# Autodesk Inventor assembly: GGC_V1
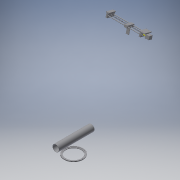
[picture p0: Inventor's stored thumbnail of the model, 180x180]
Saved by Autodesk Inventor 2016 (Build 200138000, 138)
## iProperties
Created: 2016-04-14
Part Number: GGC_V1
Document SubType Name: Assembly
Designer: rmarkowi
Author: rmarkowi
## Documents named in this file (11)
- C:\Users\rmarkowi\Documents\GGC\V1\GGC_V1.iam
- C:\Users\rmarkowi\Documents\GGC\V1\Inner Pole.ipt
- C:\Users\rmarkowi\Documents\GGC\V1\Turntable_2.ipt
- C:\Users\rmarkowi\Documents\GGC\V1\Near Gantry Bracket.ipt
- C:\Users\rmarkowi\Documents\GGC\V1\Threaded Rod.ipt
- C:\Users\rmarkowi\Documents\GGC\V1\Unthreaded Rod.ipt
- C:\Users\rmarkowi\Documents\GGC\V1\Far Gantry Bracket.ipt
- C:\Users\rmarkowi\Documents\GGC\V1\Traveller.ipt
- C:\Users\rmarkowi\Documents\GGC\V1\Threaded Rod Nut.ipt
- C:\Users\rmarkowi\Documents\GGC\V1\Threaded Rod Coupler.ipt
- C:\Users\rmarkowi\Documents\GGC\V1\NEMA23 Motor.ipt
## Components (12 placed, 10 different names)
1. Inner Pole:1
2. Turntable_2:1
3. Threaded Rod:1 — Mate:8, Mate:9, Mate:21
4. Unthreaded Rod:1 — Mate:10, Mate:11, Mate:18
5. Unthreaded Rod:2 — Mate:6, Mate:7, Mate:19, Flush:1, Mate:24
6. Near Gantry Bracket:2 — Flush:1, Flush:2, Mate:24, Mate:25, Mate:26
7. Far Gantry Bracket:1 — Mate:6, Mate:7, Mate:8, Mate:9, Mate:10, Mate:11, Flush:2
8. Traveller:1 — Mate:12, Mate:13, Mate:14, Mate:15, Mate:16, Mate:17, Mate:18, Mate:19
9. Threaded Rod Nut:1 — Mate:12, Mate:13, Mate:14
10. Threaded Rod Nut:2 — Mate:15, Mate:16, Mate:17
11. Threaded Rod Coupler:1 — Mate:21, Mate:22, Mate:23
12. NEMA23 Motor:1 — Mate:22, Mate:23, Mate:25, Mate:26
## Relationships (22: Mate 20, Flush 2)
- Mate:6: Unthreaded Rod:2 ↔ Far Gantry Bracket:1
- Mate:7: Unthreaded Rod:2 ↔ Far Gantry Bracket:1
- Mate:8: Threaded Rod:1 ↔ Far Gantry Bracket:1
- Mate:9: Threaded Rod:1 ↔ Far Gantry Bracket:1
- Mate:10: Unthreaded Rod:1 ↔ Far Gantry Bracket:1
- Mate:11: Unthreaded Rod:1 ↔ Far Gantry Bracket:1
- Mate:12: Traveller:1 ↔ Threaded Rod Nut:1
- Mate:13: Traveller:1 ↔ Threaded Rod Nut:1
- Mate:14: Traveller:1 ↔ Threaded Rod Nut:1
- Mate:15: Traveller:1 ↔ Threaded Rod Nut:2
- Mate:16: Traveller:1 ↔ Threaded Rod Nut:2
- Mate:17: Traveller:1 ↔ Threaded Rod Nut:2
- Mate:18: Unthreaded Rod:1 ↔ Traveller:1
- Mate:19: Unthreaded Rod:2 ↔ Traveller:1
- Mate:21: Threaded Rod:1 ↔ Threaded Rod Coupler:1
- Mate:22: Threaded Rod Coupler:1 ↔ NEMA23 Motor:1
- Mate:23: Threaded Rod Coupler:1 ↔ NEMA23 Motor:1
- Flush:1 (25.4 mm): Unthreaded Rod:2 ↔ Near Gantry Bracket:2
- Flush:2: Near Gantry Bracket:2 ↔ Far Gantry Bracket:1
- Mate:24: Unthreaded Rod:2 ↔ Near Gantry Bracket:2
- Mate:25: Near Gantry Bracket:2 ↔ NEMA23 Motor:1
- Mate:26: Near Gantry Bracket:2 ↔ NEMA23 Motor:1
